# Autodesk Inventor assembly: CompensationAndCombination
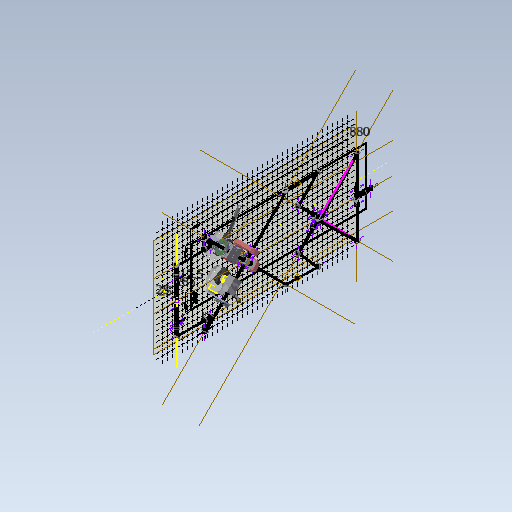
[picture p0: Inventor's stored thumbnail of the model, 512x512]
Saved by Autodesk Inventor 2020 (Build 240168000, 168)
## iProperties
Created: 2016-12-01
Part Number: CompensationAndCombination
Document SubType Name: Assembly
Designer: map
Author: map
## Documents named in this file (22)
- C:\Users\whgu0532\Documents\4Pi\4Pi-Oxford\02-CompensationAndCombination.iam
- C:\Users\whgu0532\Documents\4Pi\4Pi-Oxford\__CAVITY_AND_IMAGING_OPTICS__.iam
- C:\Users\whgu0532\Documents\4Pi\4Pi-Oxford\CVI_Shutter\CVI Melles Griot - 04RDI132 Shutter.iam
- C:\Users\whgu0532\Documents\4Pi\4Pi-Oxford\CVI_Shutter\FAB-CAM005 - Shutter Mount V2.ipt
- C:\Users\whgu0532\Documents\4Pi\4Pi-Oxford\Wedges\Wedge Mount- Upper.iam
- C:\Users\whgu0532\Documents\4Pi\4Pi-Oxford\Goniometer\M-RS65 bottom.ipt
- C:\Users\whgu0532\Documents\4Pi\4Pi-Oxford\Goniometer\M-RS65 top.ipt
- C:\Users\whgu0532\Documents\4Pi\4Pi-Oxford\Goniometer\TRA12CC.ipt
- C:\Users\whgu0532\Documents\4Pi\4Pi-Oxford\Goniometer\M-GON40-U.ipt
- C:\Users\whgu0532\Documents\4Pi\4Pi-Oxford\beam splitter cube.ipt
- C:\Users\whgu0532\Documents\4Pi\4Pi-Oxford\FAB-P0044 - Lens Mount - 40mm Upper.ipt
- C:\Users\whgu0532\Documents\4Pi\4Pi-Oxford\Wedges\FAB-P0050 - Wedge Only Mt Lower.ipt
- C:\Users\whgu0532\Documents\4Pi\4Pi-Oxford\Wedges\Thor MT1-M-Z8 Motorized Translation Stage1.ipt
- C:\Users\whgu0532\Documents\4Pi\4Pi-Oxford\MSVC3-15.ipt
- C:\Users\whgu0532\Documents\4Pi\4Pi-Oxford\Wedges\Wedge Glass1.iam
- C:\Users\whgu0532\Documents\4Pi\4Pi-Oxford\FAB-OX0003-Wedge.Lower.Baseplate.ipt
- C:\Users\whgu0532\Documents\4Pi\4Pi-Oxford\HoleGrid.ipt
- C:\Users\whgu0532\Documents\4Pi\4Pi-Oxford\FAB-OX0004-Wedge.Upper.Baseplate.ipt
- C:\Users\whgu0532\Documents\4Pi\4Pi-Oxford\FAB-OX0005-GoniometerSpacer.ipt
- C:\Users\whgu0532\Documents\4Pi\4Pi-Oxford\FAB-OX0006-GoniometerCubeMount.ipt
- C:\Users\whgu0532\Documents\4Pi\4Pi-Oxford\FAB-OX0007-LensMount40mm.Lower.Derived.ipt
- C:\Users\whgu0532\Documents\4Pi\4Pi-Oxford\FAB-OX0008-WedgeSupport.Lower.Derived.ipt
## Components (25 placed, 21 different names)
1. __CAVITY_AND_IMAGING_OPTICS__:1 [sub-assembly] — Mate:28, Tangent:1, Tangent:2, Tangent:3, Tangent:4, Tangent:5, Tangent:6, Mate:33, Mate:34, Mate:37, Mate:45, Mate:46, Flush:11, Flush:13, Flush:15, Angle:4
2. HoleGrid:1
3. CVI Melles Griot - 04RDI132 Shutter:1 [sub-assembly] — Mate:5
4. CVI Melles Griot - 04RDI132 Shutter:2 [sub-assembly] — Mate:7, Mate:8
5. FAB-CAM005 - Shutter Mount V2:1 — Mate:5, Mate:28, Mate:33, Mate:34, Mate:60
6. FAB-CAM005 - Shutter Mount V2:2 — Mate:7, Mate:8, Mate:37, Mate:58, Angle:3
7. Wedge Mount- Upper:1 [sub-assembly] — Mate:61, Mate:62, Flush:15
8. M-RS65 bottom:1 — Mate:11, Mate:12, Mate:20, Mate:21, Flush:16
9. M-RS65 top:1 — Mate:11, Mate:12, Mate:66, Insert:1, Insert:2
10. M-GON40-U:1 — Mate:18, Mate:19, Angle:4, Mate:65, Mate:67, Mate:68, Mate:69, Mate:70
11. beam splitter cube:1 — Mate:45, Mate:46, Mate:57, Mate:62, Mate:63, Mate:64
12. TRA12CC:1 — Mate:18, Mate:19
13. TRA12CC:2 — Mate:20, Mate:21
14. FAB-OX0007-LensMount40mm.Lower.Derived:1 — Tangent:1, Tangent:2, Tangent:3, Flush:9
15. FAB-P0044 - Lens Mount - 40mm Upper:2 — Tangent:4, Tangent:5, Flush:9, Tangent:6
16. FAB-P0050 - Wedge Only Mt Lower:1
17. FAB-OX0008-WedgeSupport.Lower.Derived:1 — Mate:54, Mate:55, Mate:71
18. Thor MT1-M-Z8 Motorized Translation Stage1:1 — Mate:72
19. MSVC3-15:1 — Rigid:1
20. MSVC3-15:2 — Rigid:2
21. Wedge Glass1:1 [sub-assembly] — Mate:54, Mate:55, Flush:11, Flush:13, Mate:57
22. FAB-OX0003-Wedge.Lower.Baseplate:1 — Rigid:1, Rigid:2, Mate:58, Angle:3, Flush:14, Mate:71, Mate:72
23. FAB-OX0004-Wedge.Upper.Baseplate:1 — Mate:60, Flush:14, Mate:61, Flush:16
24. FAB-OX0005-GoniometerSpacer:1 — Insert:1, Insert:2, Mate:67
25. FAB-OX0006-GoniometerCubeMount:1 — Mate:68, Mate:69, Mate:70
## Relationships (56: Mate 38, Tangent 6, Flush 6, WeldJoint 2, Angle 2, Insert 2)
- Mate:5: CVI Melles Griot - 04RDI132 Shutter:1 ↔ FAB-CAM005 - Shutter Mount V2:1
- Mate:7: CVI Melles Griot - 04RDI132 Shutter:2 ↔ FAB-CAM005 - Shutter Mount V2:2
- Mate:8: CVI Melles Griot - 04RDI132 Shutter:2 ↔ FAB-CAM005 - Shutter Mount V2:2
- Mate:11: M-RS65 bottom:1 ↔ M-RS65 top:1
- Mate:12: M-RS65 bottom:1 ↔ M-RS65 top:1
- Mate:18: M-GON40-U:1 ↔ TRA12CC:1
- Mate:19: M-GON40-U:1 ↔ TRA12CC:1
- Mate:20: M-RS65 bottom:1 ↔ TRA12CC:2
- Mate:21: M-RS65 bottom:1 ↔ TRA12CC:2
- Mate:28: __CAVITY_AND_IMAGING_OPTICS__:1 ↔ FAB-CAM005 - Shutter Mount V2:1
- Tangent:1: __CAVITY_AND_IMAGING_OPTICS__:1 ↔ FAB-OX0007-LensMount40mm.Lower.Derived:1
- Tangent:2: __CAVITY_AND_IMAGING_OPTICS__:1 ↔ FAB-OX0007-LensMount40mm.Lower.Derived:1
- Tangent:3 (-0.37 mm): __CAVITY_AND_IMAGING_OPTICS__:1 ↔ FAB-OX0007-LensMount40mm.Lower.Derived:1
- Tangent:4: __CAVITY_AND_IMAGING_OPTICS__:1 ↔ FAB-P0044 - Lens Mount - 40mm Upper:2
- Tangent:5: __CAVITY_AND_IMAGING_OPTICS__:1 ↔ FAB-P0044 - Lens Mount - 40mm Upper:2
- Flush:9: FAB-OX0007-LensMount40mm.Lower.Derived:1 ↔ FAB-P0044 - Lens Mount - 40mm Upper:2
- Tangent:6 (-0.37 mm): __CAVITY_AND_IMAGING_OPTICS__:1 ↔ FAB-P0044 - Lens Mount - 40mm Upper:2
- Mate:33: __CAVITY_AND_IMAGING_OPTICS__:1 ↔ FAB-CAM005 - Shutter Mount V2:1
- Mate:34: __CAVITY_AND_IMAGING_OPTICS__:1 ↔ FAB-CAM005 - Shutter Mount V2:1
- Mate:37: __CAVITY_AND_IMAGING_OPTICS__:1 ↔ FAB-CAM005 - Shutter Mount V2:2
- Mate:45: __CAVITY_AND_IMAGING_OPTICS__:1 ↔ beam splitter cube:1
- Mate:46: __CAVITY_AND_IMAGING_OPTICS__:1 ↔ beam splitter cube:1
- [Mate]: FAB-P0050 - Wedge Only Mt Lower:1 ↔ Thor MT1-M-Z8 Motorized Translation Stage1:1
- [Mate]: FAB-P0050 - Wedge Only Mt Lower:1 ↔ Thor MT1-M-Z8 Motorized Translation Stage1:1
- [Mate]: FAB-P0050 - Wedge Only Mt Lower:1 ↔ Thor MT1-M-Z8 Motorized Translation Stage1:1
- [Mate]: FAB-P0050 - Wedge Only Mt Lower:1 ↔ Wedge Glass1:1
- [Mate]: FAB-P0050 - Wedge Only Mt Lower:1 ↔ Wedge Glass1:1
- Mate:54 (0.006 mm): FAB-OX0008-WedgeSupport.Lower.Derived:1 ↔ Wedge Glass1:1
- Mate:55: FAB-OX0008-WedgeSupport.Lower.Derived:1 ↔ Wedge Glass1:1
- Flush:11: __CAVITY_AND_IMAGING_OPTICS__:1 ↔ Wedge Glass1:1
- Flush:13: __CAVITY_AND_IMAGING_OPTICS__:1 ↔ Wedge Glass1:1
- Mate:57 (85 mm): beam splitter cube:1 ↔ Wedge Glass1:1
- Rigid:1 [WeldJoint]: MSVC3-15:1 ↔ FAB-OX0003-Wedge.Lower.Baseplate:1
- Rigid:2 [WeldJoint]: MSVC3-15:2 ↔ FAB-OX0003-Wedge.Lower.Baseplate:1
- Mate:58: FAB-CAM005 - Shutter Mount V2:2 ↔ FAB-OX0003-Wedge.Lower.Baseplate:1
- Angle:3 (0 deg): FAB-CAM005 - Shutter Mount V2:2 ↔ FAB-OX0003-Wedge.Lower.Baseplate:1
- [Mate]: Wedge Mount- Upper:1 ↔ FAB-OX0004-Wedge.Upper.Baseplate:1
- Mate:60: FAB-CAM005 - Shutter Mount V2:1 ↔ FAB-OX0004-Wedge.Upper.Baseplate:1
- Flush:14: FAB-OX0003-Wedge.Lower.Baseplate:1 ↔ FAB-OX0004-Wedge.Upper.Baseplate:1
- Mate:61: Wedge Mount- Upper:1 ↔ FAB-OX0004-Wedge.Upper.Baseplate:1
- Mate:62 (85 mm): Wedge Mount- Upper:1 ↔ beam splitter cube:1
- Flush:15: __CAVITY_AND_IMAGING_OPTICS__:1 ↔ Wedge Mount- Upper:1
- Flush:16: M-RS65 bottom:1 ↔ FAB-OX0004-Wedge.Upper.Baseplate:1
- Angle:4 (270 deg): __CAVITY_AND_IMAGING_OPTICS__:1 ↔ M-GON40-U:1
- Mate:63: beam splitter cube:1
- Mate:64: beam splitter cube:1
- Mate:65: M-GON40-U:1
- Mate:66: M-RS65 top:1
- Insert:1: M-RS65 top:1 ↔ FAB-OX0005-GoniometerSpacer:1
- Insert:2: M-RS65 top:1 ↔ FAB-OX0005-GoniometerSpacer:1
- Mate:67: M-GON40-U:1 ↔ FAB-OX0005-GoniometerSpacer:1
- Mate:68: M-GON40-U:1 ↔ FAB-OX0006-GoniometerCubeMount:1
- Mate:69: M-GON40-U:1 ↔ FAB-OX0006-GoniometerCubeMount:1
- Mate:70: M-GON40-U:1 ↔ FAB-OX0006-GoniometerCubeMount:1
- Mate:71: FAB-OX0008-WedgeSupport.Lower.Derived:1 ↔ FAB-OX0003-Wedge.Lower.Baseplate:1
- Mate:72: Thor MT1-M-Z8 Motorized Translation Stage1:1 ↔ FAB-OX0003-Wedge.Lower.Baseplate:1
## Named parameters: d80_d20 = 0 mm, d82_d16 = 0.006 mm, d85_d3 = 0 mm, d86_d4 = 0 mm, d87_d5 = 0 mm, d88_d6 = 0 mm, d89_d7 = 0 mm
